# Autodesk Inventor assembly: slide assembly
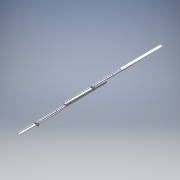
[picture p0: Inventor's stored thumbnail of the model, 180x180]
Saved by Autodesk Inventor 2019 (Build 230136000, 136)
## iProperties
Created: 2019-05-04
Part Number: slide assembly
Document SubType Name: Assembly
Designer: Delta
Author: Delta
## Documents named in this file (4)
- C:\Robotics\2019-20_CAD\offseason\random ideas\slides\slide assembly.iam
- C:\Robotics\2019-20_CAD\offseason\random ideas\slides\SAR330.iam
- C:\Robotics\2019-20_CAD\offseason\random ideas\slides\slide conector.ipt
- C:\Robotics\2019-20_CAD\Linear Slides\Pulley assembly.iam
## Components (5 placed, 3 different names)
1. SAR330:1 [sub-assembly] — Mate:1, Mate:2, Mate:3, Mate:15, Mate:16, Mate:17
2. SAR330:2 [sub-assembly] — Mate:4, Mate:5, Mate:6, Mate:13, Mate:14, Flush:4
3. slide conector:1 — Mate:1, Mate:2, Mate:3, Mate:4, Mate:5, Mate:6
4. Pulley assembly:1 [sub-assembly] — Mate:13, Mate:14, Flush:4
5. Pulley assembly:3 [sub-assembly] — Mate:15, Mate:16, Mate:17
## Relationships (12: Mate 11, Flush 1)
- Mate:1: SAR330:1 ↔ slide conector:1
- Mate:2: SAR330:1 ↔ slide conector:1
- Mate:3: SAR330:1 ↔ slide conector:1
- Mate:4: SAR330:2 ↔ slide conector:1
- Mate:5: SAR330:2 ↔ slide conector:1
- Mate:6: SAR330:2 ↔ slide conector:1
- Mate:13: SAR330:2 ↔ Pulley assembly:1
- Mate:14: SAR330:2 ↔ Pulley assembly:1
- Flush:4: SAR330:2 ↔ Pulley assembly:1
- Mate:15: SAR330:1 ↔ Pulley assembly:3
- Mate:16: SAR330:1 ↔ Pulley assembly:3
- Mate:17: SAR330:1 ↔ Pulley assembly:3
